# Autodesk Inventor assembly: 276-2016
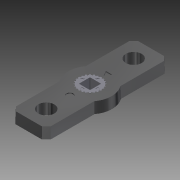
[picture p0: Inventor's stored thumbnail of the model, 180x180]
Saved by Autodesk Inventor 2013 (Build 170138000, 138)
## iProperties
Company: Autodesk Inc.
Category: Motion
Created: 2012-04-11
Part Number: 276-2016
Document SubType Name: Assembly
Designer: Autodesk Inc.
Catalog Web Link: http://www.vexrobotics.com/276-2016.html
Vendor: VEX
Author: Autodesk Inc.
## Documents named in this file (3)
- C:\Data Folder\VEX 2012\VEX KOP Uploads\2013\Metric\Motion\Lock Bar.iam
- C:\Data Folder\VEX 2012\VEX KOP Uploads\2013\Metric\Motion\Components\Shaft Lock Bar.ipt
- C:\Data Folder\VEX 2012\VEX KOP Uploads\2013\Metric\Motion\Components\Shaft Lock Bar Insert.ipt
## Components (2 placed, 2 different names)
1. Shaft Lock Bar:1 — Flush:1
2. Shaft Lock Bar Insert:1 — Flush:1
## Relationships (1: Flush 1)
- Flush:1: Shaft Lock Bar:1 ↔ Shaft Lock Bar Insert:1
